# Autodesk Inventor assembly: hallEffectSensorAssembly
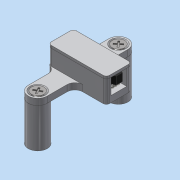
[picture p0: Inventor's stored thumbnail of the model, 180x180]
Saved by Autodesk Inventor 2017.3 (Build 213256000, 256)
## iProperties
Created: 2018-08-31
Part Number: hallEffectSensorAssembly
Document SubType Name: Assembly
Designer: Derek Wider
Author: Derek Wider
## Documents named in this file (6)
- G:\Projects\Submarine\Submarine-project\CAD\aft\encoder\hallEffectSensorAssembly.iam
- G:\Projects\Submarine\Submarine-project\CAD\aft\encoder\HallEffectSensorCase.ipt
- G:\Projects\Submarine\Submarine-project\CAD\aft\encoder\HallEffectSensorCaseLid.ipt
- G:\Projects\Submarine\Submarine-project\CAD\aft\encoder\photoTransistorStandoff.ipt
- G:\Projects\Submarine\Submarine-project\CAD\common\screws\flatPlasticScrewSmall.ipt
- G:\Projects\Submarine\Submarine-project\CAD\aft\encoder\HallEffectSensorBentPins.ipt
## Components (7 placed, 5 different names)
1. HallEffectSensorCase:1 — Mate:4, Flush:1, Flush:2, Mate:5, Mate:6, Mate:7, Mate:8, Mate:9, Mate:10, Flush:3, Flush:4
2. HallEffectSensorCaseLid:1 — Mate:1, Mate:2, Mate:3, Mate:4, Flush:1, Flush:2
3. photoTransistorStandoff:1 — Mate:5, Mate:6
4. photoTransistorStandoff:2 — Mate:7, Mate:8
5. flatPlasticScrewSmall:1 — Mate:9, Flush:4
6. flatPlasticScrewSmall:2 — Mate:10, Flush:3
7. HallEffectSensorBentPins:1 — Mate:1, Mate:2, Mate:3
## Relationships (14: Mate 10, Flush 4)
- Mate:1: HallEffectSensorCaseLid:1 ↔ HallEffectSensorBentPins:1
- Mate:2 (-0.635 mm): HallEffectSensorCaseLid:1 ↔ HallEffectSensorBentPins:1
- Mate:3 (0.508 mm): HallEffectSensorCaseLid:1 ↔ HallEffectSensorBentPins:1
- Mate:4: HallEffectSensorCase:1 ↔ HallEffectSensorCaseLid:1
- Flush:1: HallEffectSensorCase:1 ↔ HallEffectSensorCaseLid:1
- Flush:2: HallEffectSensorCase:1 ↔ HallEffectSensorCaseLid:1
- Mate:5: HallEffectSensorCase:1 ↔ photoTransistorStandoff:1
- Mate:6: HallEffectSensorCase:1 ↔ photoTransistorStandoff:1
- Mate:7: HallEffectSensorCase:1 ↔ photoTransistorStandoff:2
- Mate:8: HallEffectSensorCase:1 ↔ photoTransistorStandoff:2
- Mate:9: HallEffectSensorCase:1 ↔ flatPlasticScrewSmall:1
- Mate:10: HallEffectSensorCase:1 ↔ flatPlasticScrewSmall:2
- Flush:3: HallEffectSensorCase:1 ↔ flatPlasticScrewSmall:2
- Flush:4: HallEffectSensorCase:1 ↔ flatPlasticScrewSmall:1
